# Autodesk Inventor assembly: Rueda con transmision
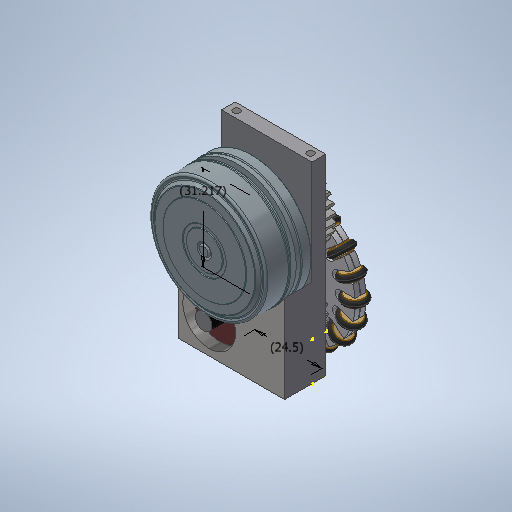
[picture p0: Inventor's stored thumbnail of the model, 512x512]
Saved by Autodesk Inventor 2025.1 (Build 291241000, 241)
## iProperties
Part Number: Rueda con transmision
Material: Generisch
Document SubType Name: Assembly
Designer: stefa
Mass: 192.049 g
Surface Area: 432.638 cm^2
Volume: 68.0143 cm^3
Density: 2.82366 g/cm^3
Author: stefa
## Documents named in this file (8)
- C:\Users\paeze\Downloads\Base_Ruedas\Rueda con transmision.iam
- C:\Users\paeze\hardware\pasta\mechanics\Wheel\WH_Motormount_right.ipt
- C:\Users\paeze\Downloads\Base_Ruedas\387266-ec45fl-30w-a-kabel\387266_ec45fl_30w_a_kabel\387266_ec45fl_30w_a_kabel\387266_ec45fl_30w_a_kabel.ipt
- C:\Users\paeze\Downloads\Base_Ruedas\gtf-robots-50mm-omniwheel-1.snapshot.2\GTF Robots 50mm Wheel v4\GTF Robots 50mm Wheel v4\GTF Robots 50mm Wheel v4.ipt
- C:\Users\paeze\Downloads\Base_Ruedas\Eje.ipt
- C:\Users\paeze\Downloads\Base_Ruedas\Engraneeeee.ipt
- C:\Users\paeze\Downloads\Base_Ruedas\Engraneeee.ipt
- C:\Users\paeze\Downloads\Base_Ruedas\28_08\Ruleman.ipt
## Components (7 placed, 7 different names)
1. WH_Motormount_right:1 — Fluchtend:1, Fluchtend:2, Fluchtend:3, Rotational:1, Rigid:6, Rotational:2
2. 387266_ec45fl_30w_a_kabel:1 — Rotational:1, Rigid:5
3. GTF Robots 50mm Wheel v4:1
4. Eje:1 — Rigid:6
5. Spur Gear1:1 — Rigid:5
6. Spur Gear2:1
7. Ruleman:1 — Rotational:2
## Relationships (7: Flush 3, RevoluteJoint 2, WeldJoint 2)
- Fluchtend:1 [Flush]: WH_Motormount_right:1
- Fluchtend:2 [Flush]: WH_Motormount_right:1
- Fluchtend:3 [Flush]: WH_Motormount_right:1
- Rotational:1 [RevoluteJoint]: WH_Motormount_right:1 ↔ 387266_ec45fl_30w_a_kabel:1
- Rigid:5 [WeldJoint]: 387266_ec45fl_30w_a_kabel:1 ↔ Spur Gear1:1
- Rigid:6 [WeldJoint] (-12 mm): WH_Motormount_right:1 ↔ Eje:1
- Rotational:2 [RevoluteJoint]: WH_Motormount_right:1 ↔ Ruleman:1
